# Autodesk Inventor assembly: masih belum
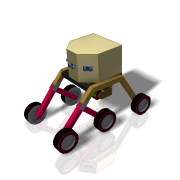
[picture p0: Inventor's stored thumbnail of the model, 180x180]
Saved by Autodesk Inventor 2018 (Build 220112000, 112)
## iProperties
Created: 2019-12-19
Part Number: masih belum
Document SubType Name: Assembly
Designer: Ibnu
Author: Ibnu
## Documents named in this file (9)
- C:\Users\Ibnu\Documents\Inventor\ROCKER BOGIE ROBOT\masih belum.iam
- C:\Users\Ibnu\Documents\Inventor\ROCKER BOGIE ROBOT\bodi metal.ipt
- C:\Users\Ibnu\Documents\Inventor\ROCKER BOGIE ROBOT\plat sim.ipt
- C:\Users\Ibnu\Documents\Inventor\ROCKER BOGIE ROBOT\l almini.ipt
- C:\Users\Ibnu\Documents\Inventor\ROCKER BOGIE ROBOT\roda sim.ipt
- C:\Users\Ibnu\Documents\Inventor\ROCKER BOGIE ROBOT\sambung kotak.ipt
- C:\Users\Ibnu\Documents\Inventor\ROCKER BOGIE ROBOT\bodyy.ipt
- C:\Users\Ibnu\Documents\Inventor\ROCKER BOGIE ROBOT\gopro.iam
- C:\Users\Ibnu\Documents\Inventor\ROCKER BOGIE ROBOT\Ultrasonic HCSR04.ipt
## Components (20 placed, 8 different names)
1. bodi metal:1 — Insert:6, Mate:2, Mate:3, Mate:4, Mate:13, Mate:14, Mate:15, Mate:16, Mate:17, Mate:18
2. plat sim:1 — Mate:14, Mate:15, Mate:16
3. plat sim:2 — Mate:13, Mate:17, Mate:18, Insert:12
4. l almini:1 — Insert:2, Insert:3, Insert:12
5. roda sim:1 — Insert:3
6. roda sim:2 — Insert:6
7. roda sim:3 — Insert:2
8. sambung kotak:1 — Mate:2, Mate:3, Mate:4, Insert:7, Mate:11, Mate:12
9. bodi metal:2 — Insert:7, Mate:5, Mate:6, Mate:7, Mate:8, Mate:9, Mate:10, Insert:11
10. plat sim:3 — Mate:8, Mate:9, Mate:10, Insert:8
11. plat sim:4 — Mate:5, Mate:6, Mate:7
12. roda sim:4 — Insert:9
13. roda sim:5 — Insert:10
14. roda sim:6 — Insert:11
15. l almini:2 — Insert:8, Insert:9, Insert:10
16. bodyy:1 — Mate:11, Mate:12, Mate:19, Mate:20, Mate:21, Mate:22, Mate:23, Mate:24, Mate:25, Mate:26, Mate:27, Mate:28
17. gopro:2 [sub-assembly] — Mate:19, Mate:20, Mate:21
18. Ultrasonic HCSR04:1 — Mate:22, Mate:23, Mate:24
19. Ultrasonic HCSR04:2 — Mate:27, Mate:28
20. Ultrasonic HCSR04:3 — Mate:25, Mate:26
## Relationships (36: Mate 27, Insert 9)
- Insert:2 (15 mm): l almini:1 ↔ roda sim:3
- Insert:3 (15 mm): l almini:1 ↔ roda sim:1
- Insert:6 (15 mm): bodi metal:1 ↔ roda sim:2
- Mate:2: bodi metal:1 ↔ sambung kotak:1
- Mate:3: bodi metal:1 ↔ sambung kotak:1
- Mate:4: bodi metal:1 ↔ sambung kotak:1
- Insert:7: sambung kotak:1 ↔ bodi metal:2
- Mate:5: bodi metal:2 ↔ plat sim:4
- Mate:6: bodi metal:2 ↔ plat sim:4
- Mate:7: bodi metal:2 ↔ plat sim:4
- Mate:8: bodi metal:2 ↔ plat sim:3
- Mate:9: bodi metal:2 ↔ plat sim:3
- Mate:10: bodi metal:2 ↔ plat sim:3
- Insert:8: plat sim:3 ↔ l almini:2
- Insert:9 (15 mm): roda sim:4 ↔ l almini:2
- Insert:10 (15 mm): roda sim:5 ↔ l almini:2
- Insert:11 (15 mm): bodi metal:2 ↔ roda sim:6
- Mate:11: sambung kotak:1 ↔ bodyy:1
- Mate:12: sambung kotak:1 ↔ bodyy:1
- Mate:13: bodi metal:1 ↔ plat sim:2
- Mate:14: bodi metal:1 ↔ plat sim:1
- Mate:15: bodi metal:1 ↔ plat sim:1
- Mate:16: bodi metal:1 ↔ plat sim:1
- Mate:17: bodi metal:1 ↔ plat sim:2
- Mate:18: bodi metal:1 ↔ plat sim:2
- Insert:12: plat sim:2 ↔ l almini:1
- Mate:19: bodyy:1 ↔ gopro:2
- Mate:20: bodyy:1 ↔ gopro:2
- Mate:21: bodyy:1 ↔ gopro:2
- Mate:22: bodyy:1 ↔ Ultrasonic HCSR04:1
- Mate:23: bodyy:1 ↔ Ultrasonic HCSR04:1
- Mate:24: bodyy:1 ↔ Ultrasonic HCSR04:1
- Mate:25: bodyy:1 ↔ Ultrasonic HCSR04:3
- Mate:26: bodyy:1 ↔ Ultrasonic HCSR04:3
- Mate:27: bodyy:1 ↔ Ultrasonic HCSR04:2
- Mate:28: bodyy:1 ↔ Ultrasonic HCSR04:2
